# Autodesk Inventor assembly: w_cbs1240
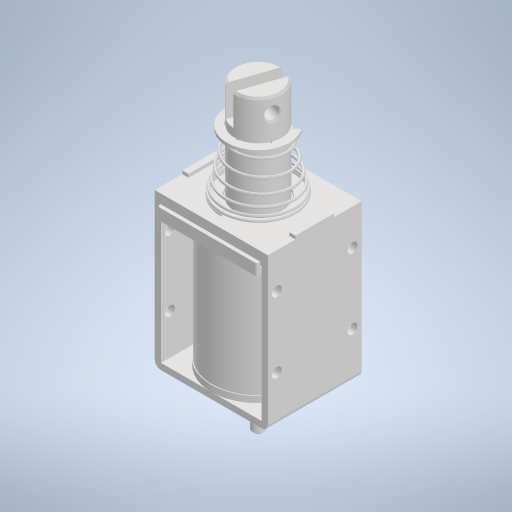
[picture p0: Inventor's stored thumbnail of the model, 512x512]
Saved by Autodesk Inventor 2023 (Build 270158000, 158)
## iProperties
Company: Hewlett-Packard Company
Created: 2014-07-25
Part Number: w_cbs1240
Description: STEP AP203
Document SubType Name: Assembly
Designer: blueh
Title: w_cbs1240.STEP
Author: jiba
Revision Number: ANY
Sending System: SolidWorks 2014
Preprocessor: SwSTEP 2.0
## Documents named in this file (4)
- C:\Users\blueh\OneDrive - Kyushu University\2023NHK_RR_2ndvid\000_parts_zegi\CBS1240w_cbs1240.iam
- C:\Users\blueh\OneDrive - Kyushu University\2023NHK_RR_2ndvid\000_parts_zegi\CBS1240Part7^w_cbs1240.ipt
- C:\Users\blueh\OneDrive - Kyushu University\2023NHK_RR_2ndvid\000_parts_zegi\CBS1240Part1^w_cbs1240_pl.ipt
- C:\Users\blueh\OneDrive - Kyushu University\2023NHK_RR_2ndvid\000_parts_zegi\CBS1240w_21240081.ipt
## Components (3 placed, 3 different names)
1. Part7^w_cbs1240_1 — 円柱状:1
2. Part1^w_cbs1240_pl_2 — 円柱状:1
3. w_21240081_3
## Relationships (1: CylindricalJoint 1)
- 円柱状:1 [CylindricalJoint]: Part7^w_cbs1240_1 ↔ Part1^w_cbs1240_pl_2
